# Autodesk Inventor assembly: battery_assm
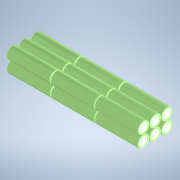
[picture p0: Inventor's stored thumbnail of the model, 180x180]
Saved by Autodesk Inventor 2020 (Build 240168000, 168)
## iProperties
Created: 2020-06-07
Part Number: battery_assm
Document SubType Name: Assembly
Designer: Abhinav Roy
Author: Abhinav Roy
## iProperties of the stored document battery case.ipt
Created: 2016-07-30
Part Number: battery case
Material: SOLIDWORKS Materials|Nylon 101
Document SubType Name: Modeling
Designer: Abhinav Roy
Density: 1.15 g/cm^3
Appearance: 171,255,127
Sending System: SolidWorks 2016
Last Author: sys_admin
Last Saved: 2016-09-19
Author: Abhinav Roy
## iProperties of the stored document 18650 battery.iam
Created: 2016-07-30
Part Number: 18650 battery
Document SubType Name: Assembly
Designer: Abhinav Roy
Sending System: SolidWorks 2016
Last Author: sys_admin
Last Saved: 2016-07-30
Author: Abhinav Roy
## iProperties of the stored document battery washer.ipt
Created: 2016-07-30
Part Number: battery washer
Material: SOLIDWORKS Materials|ABS
Document SubType Name: Modeling
Designer: Abhinav Roy
Density: 1.02 g/cm^3
Appearance: 255,255,255
Sending System: SolidWorks 2016
Last Author: sys_admin
Last Saved: 2016-08-06
Author: Abhinav Roy
## iProperties of the stored document battery terminal +.ipt
Created: 2016-07-30
Part Number: battery terminal +
Material: SOLIDWORKS Materials|Nickel
Document SubType Name: Modeling
Designer: Abhinav Roy
Density: 8.5 g/cm^3
Appearance: 255,250,247
Sending System: SolidWorks 2016
Last Author: sys_admin
Last Saved: 2016-07-30
Author: Abhinav Roy
## iProperties of the stored document battery terminal -.ipt
Created: 2016-07-30
Part Number: battery terminal -
Material: SOLIDWORKS Materials|Nickel
Document SubType Name: Modeling
Designer: Abhinav Roy
Density: 8.5 g/cm^3
Appearance: 192,192,192
Sending System: SolidWorks 2016
Last Author: sys_admin
Last Saved: 2016-09-19
Author: Abhinav Roy
## Documents named in this file (12)
- D:\Mopping_Robot\cad\V1.0\battery_assm.iam
- **D:\Mopping_Robot\cad\V1.0\battery_assm.iam*LocalDocs*xAaaaagcaAaaaaaaaAaaaqh23Xb*18650 battery.iam
- **D:\Mopping_Robot\cad\V1.0\stl_files\battery_assm.iam*LocalDocs*xAaaaahbaAaaaaaaaAaaaa4mdZg*battery case.ipt
- **D:\Mopping_Robot\cad\V1.0\stl_files\battery_assm.iam*LocalDocs*xAaaaagcaAaaaaaaaAaaaqh23Xb*18650 battery.iam
- **D:\Mopping_Robot\cad\V1.0\stl_files\battery_assm.iam*LocalDocs*xAaaaqsaaAaaaaaaaAaaaaadzOd*battery terminal -.ipt
- **D:\Mopping_Robot\cad\V1.0\stl_files\battery_assm.iam*LocalDocs*xAaaaqlcaAaaaaaaaAaaaq1wfPh*battery washer.ipt
- **D:\Mopping_Robot\cad\V1.0\stl_files\battery_assm.iam*LocalDocs*xAaaaqcaaAaaaaaaaAaaaa3qu2g*battery terminal +.ipt
- D:\Mopping_Robot\cad\V1.0\panasonic-ncr18650b-1.snapshot.5\18650 battery.SLDASM
- D:\Mopping_Robot\cad\V1.0\panasonic-ncr18650b-1.snapshot.5\battery case.SLDPRT
- D:\Mopping_Robot\cad\V1.0\panasonic-ncr18650b-1.snapshot.5\battery terminal +.SLDPRT
- D:\Mopping_Robot\cad\V1.0\panasonic-ncr18650b-1.snapshot.5\battery terminal -.SLDPRT
- D:\Mopping_Robot\cad\V1.0\panasonic-ncr18650b-1.snapshot.5\battery washer.SLDPRT
## Components (18 placed, 1 different names)
1. 18650 battery:1 [sub-assembly]
2. 18650 battery:4 [sub-assembly]
3. 18650 battery:5 [sub-assembly]
4. 18650 battery:6 [sub-assembly]
5. 18650 battery:7 [sub-assembly]
6. 18650 battery:8 [sub-assembly]
7. 18650 battery:9 [sub-assembly]
8. 18650 battery:10 [sub-assembly]
9. 18650 battery:11 [sub-assembly]
10. 18650 battery:12 [sub-assembly]
11. 18650 battery:13 [sub-assembly]
12. 18650 battery:14 [sub-assembly]
13. 18650 battery:15 [sub-assembly]
14. 18650 battery:16 [sub-assembly]
15. 18650 battery:17 [sub-assembly]
16. 18650 battery:18 [sub-assembly]
17. 18650 battery:19 [sub-assembly]
18. 18650 battery:20 [sub-assembly]
## Component patterns: (2 elements), (9 elements, first: 18650 battery:1), Component Pattern 1:2 (9 elements)
